# Autodesk Inventor assembly: FEAandWelding
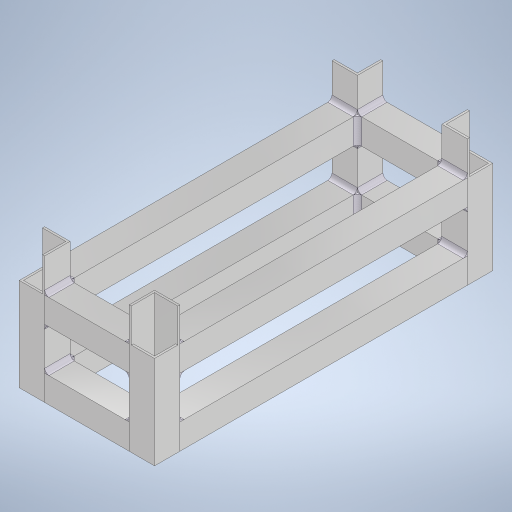
[picture p0: Inventor's stored thumbnail of the model, 512x512]
Saved by Autodesk Inventor 2023 (Build 270158000, 158)
## iProperties
Created: 2022-09-19
Part Number: FEAandWelding
Document SubType Name: Weldment
Designer: seene
Weld Material: Aluminum 6061, Welded
Author: seene
## Documents named in this file (9)
- C:\Users\seene\Desktop\Stony Brook\SBRT\RoboRescue\Chassis\Frame\FEAandWelding.iam
- C:\Users\seene\Desktop\Stony Brook\SBRT\RoboRescue\Chassis\Frame\testRoboRescue_Chassis_Frame.iam
- RoboRescue_Chassis_Frame.iam
- C:\Users\seene\Desktop\Stony Brook\SBRT\RoboRescue\Chassis\Frame\FEAandWelding\AIP\FEA\e3ixfb5nk.fins
- C:\Users\seene\Desktop\Stony Brook\SBRT\RoboRescue\Chassis\Frame\FEAandWelding\AIP\FEA\e3ixfb5nk.fsat
- C:\Users\seene\Desktop\Stony Brook\SBRT\RoboRescue\Chassis\Frame\FEAandWelding\AIP\FEA\e3ixfb5nk.ftes
- C:\Users\seene\Desktop\Stony Brook\SBRT\RoboRescue\Chassis\Frame\FEAandWelding\AIP\FEA\e3ixfb5nk.fwiz
- C:\Users\seene\Desktop\Stony Brook\SBRT\RoboRescue\Chassis\Frame\FEAandWelding\AIP\FEA\e3ixfb5vk.fmsh
- C:\Users\seene\Desktop\Stony Brook\SBRT\RoboRescue\Chassis\Frame\FEAandWelding\AIP\FEA\e3ixfb5vl.fres
## Components (1 placed, 1 different names)
1. RoboRescue_Chassis_Frame:1 [sub-assembly]
## Named parameters: sa_0 = 17792.9
note: some values were not read from the file. Shown as the stored number, unit unknown: "sa_0".
